# Autodesk Inventor assembly: A2017_T5_11
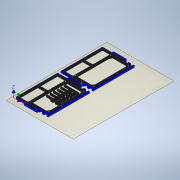
[picture p0: Inventor's stored thumbnail of the model, 180x180]
Saved by Autodesk Inventor 2022 (Build 260153000, 153)
## iProperties
Created: 2022-09-28
Part Number: A2017_T5_11
Document SubType Name: Assembly
Designer: Masato
Author: Masato
## Documents named in this file (4)
- C:\Users\ヨコオリク\Documents\CITBrains\SUSTAINA-OP\Cam\A2017_T5\A2017_T5_11.iam
- C:\Users\ヨコオリク\Documents\CITBrains\SUSTAINA-OP\Cam\DisposableBoard.ipt
- C:\Users\ヨコオリク\Documents\CITBrains\SUSTAINA-OP\UpperBody\Cockpit\Cockpit_trunk_lower_side_frame_stopper.ipt
- C:\Users\ヨコオリク\Documents\CITBrains\SUSTAINA-OP\UpperBody\Cockpit\Cockpit_circuit_board_frame.ipt
## Components (9 placed, 3 different names)
1. DisposableBoard:1 — フラッシュ:1, フラッシュ:2, フラッシュ:3, フラッシュ:4, フラッシュ:5, フラッシュ:6
2. Cockpit_circuit_board_frame:1 — メイト:1, フラッシュ:5, フラッシュ:6, メイト:3, メイト:4
3. Cockpit_circuit_board_frame:2
4. Cockpit_trunk_lower_side_frame_stopper:1 — メイト:2, メイト:3, メイト:4
5. Cockpit_trunk_lower_side_frame_stopper:2
6. Cockpit_trunk_lower_side_frame_stopper:3
7. Cockpit_trunk_lower_side_frame_stopper:4
8. Cockpit_trunk_lower_side_frame_stopper:5
9. Cockpit_trunk_lower_side_frame_stopper:6
## Component patterns: (2 elements, first: Cockpit_circuit_board_frame:1), (6 elements, first: Cockpit_trunk_lower_side_frame_stopper:1)
## Relationships (10: Flush 6, Mate 4)
- フラッシュ:1 [Flush]: DisposableBoard:1
- フラッシュ:2 [Flush]: DisposableBoard:1
- フラッシュ:3 [Flush]: DisposableBoard:1
- フラッシュ:4 [Flush]: DisposableBoard:1
- メイト:1 [Mate]: Cockpit_circuit_board_frame:1
- メイト:2 [Mate]: Cockpit_trunk_lower_side_frame_stopper:1
- フラッシュ:5 [Flush] (2 mm): DisposableBoard:1 ↔ Cockpit_circuit_board_frame:1
- フラッシュ:6 [Flush] (2 mm): DisposableBoard:1 ↔ Cockpit_circuit_board_frame:1
- メイト:3 [Mate] (10 mm): Cockpit_circuit_board_frame:1 ↔ Cockpit_trunk_lower_side_frame_stopper:1
- メイト:4 [Mate] (3 mm): Cockpit_circuit_board_frame:1 ↔ Cockpit_trunk_lower_side_frame_stopper:1
